# Autodesk Inventor assembly: 换向阀
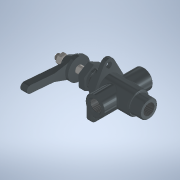
[picture p0: Inventor's stored thumbnail of the model, 180x180]
Saved by Autodesk Inventor 2022 (Build 260153000, 153)
## iProperties
Created: 2023-01-26
Part Number: 换向阀
Document SubType Name: Assembly
Designer: Lzy18
Author: Lzy18
## Documents named in this file (8)
- C:\Users\Lzy18\Desktop\第二次培训\换向阀.iam
- C:\Users\Lzy18\Desktop\第二次培训\1-阀体.ipt
- C:\Users\Lzy18\Desktop\第二次培训\2-阀门.ipt
- C:\Users\Lzy18\Desktop\第二次培训\3-锁紧螺母.ipt
- C:\Users\Lzy18\Desktop\第二次培训\7-填料.ipt
- C:\Users\Lzy18\Desktop\第二次培训\4-手柄.ipt
- C:\Users\Lzy18\Desktop\第二次培训\5-垫圈.ipt
- C:\Users\Lzy18\Desktop\第二次培训\6-螺母.ipt
## Components (7 placed, 7 different names)
1. 1-阀体:1 — 配合:4, 配合:15
2. 2-阀门:1 — 配合:8, 配合:9, 配合:10, 配合:11, 配合:12, 配合:13, 插入:1
3. 3-锁紧螺母:1 — 配合:4, 配合:5, 配合:6
4. 7-填料:1 — 表面齐平:1, 配合:5, 配合:6, 插入:1, 配合:15
5. 4-手柄:1 — 配合:8, 配合:9, 配合:10
6. 5-垫圈:1 — 配合:11, 配合:12, 配合:14
7. 6-螺母:1 — 配合:13, 配合:14
## Relationships (13: Mate 11, Flush 1, Insert 1)
- 配合:4 [Mate] (7 mm): 1-阀体:1 ↔ 3-锁紧螺母:1
- 表面齐平:1 [Flush]: 7-填料:1
- 配合:5 [Mate]: 3-锁紧螺母:1 ↔ 7-填料:1
- 配合:6 [Mate]: 3-锁紧螺母:1 ↔ 7-填料:1
- 配合:8 [Mate]: 2-阀门:1 ↔ 4-手柄:1
- 配合:9 [Mate]: 2-阀门:1 ↔ 4-手柄:1
- 配合:10 [Mate]: 2-阀门:1 ↔ 4-手柄:1
- 配合:11 [Mate]: 2-阀门:1 ↔ 5-垫圈:1
- 配合:12 [Mate]: 2-阀门:1 ↔ 5-垫圈:1
- 配合:13 [Mate]: 2-阀门:1 ↔ 6-螺母:1
- 配合:14 [Mate]: 5-垫圈:1 ↔ 6-螺母:1
- 插入:1 [Insert]: 2-阀门:1 ↔ 7-填料:1
- 配合:15 [Mate]: 1-阀体:1 ↔ 7-填料:1
